# Autodesk Inventor assembly: servo grab
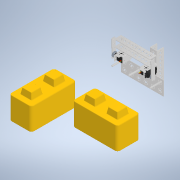
[picture p0: Inventor's stored thumbnail of the model, 180x180]
Saved by Autodesk Inventor 2020 (Build 240168000, 168)
## iProperties
Created: 2019-09-14
Part Number: servo grab
Document SubType Name: Assembly
Designer: tbloo
Author: tbloo
## Documents named in this file (9)
- D:\Documents\GitHub\AO_Robotics\CAD\Projects\Timothy Bloot\servo grab.iam
- D:\Documents\GitHub\AO_Robotics\CAD\Parts Kits\FTC Tetrix KOP Organized (7-24-19)\Stand-off posts\Tetrix_39103.ipt
- D:\Documents\GitHub\AO_Robotics\CAD\Parts Kits\FTC Tetrix KOP Organized (7-24-19)\Frame Hardware\Tetrix_39073.ipt
- D:\Documents\GitHub\AO_Robotics\CAD\Skystone Field\1x2 Block v2.ipt
- D:\Documents\GitHub\AO_Robotics\CAD\Parts Kits\FTC Tetrix KOP Organized (7-24-19)\Servo\Tetrix_39060.ipt
- D:\Documents\GitHub\AO_Robotics\CAD\Parts Kits\FTC Tetrix KOP Organized (7-24-19)\Servo\Tetrix_39197_Servo.ipt
- D:\Documents\GitHub\AO_Robotics\CAD\Parts Kits\FTC Tetrix KOP Organized (7-24-19)\Frame Hardware\Tetrix_39067.ipt
- D:\Documents\GitHub\AO_Robotics\CAD\Projects\Timothy Bloot\Tetrix_3907-5.ipt
- D:\Documents\GitHub\AO_Robotics\CAD\Parts Kits\FTC Tetrix KOP Organized (7-24-19)\Servo\Tetrix_39197_Metal_Horn.ipt
## Components (16 placed, 8 different names)
1. Tetrix_39103:1 — Rigid:8
2. Tetrix_39103:2 — Rigid:2
3. Tetrix_39103:3 — Rigid:1
4. Tetrix_39073:1 — Rigid:1, Rigid:2, Rigid:8, Rigid:9
5. 1x2 Block v2:1
6. Tetrix_39060:1 — Rigid:7, Rigid:17
7. Tetrix_39197_Servo:1 — Rigid:7, Rotational:1
8. 1x2 Block v2:2
9. Tetrix_39067:2 — Rigid:9, Rigid:19
10. Tetrix_39060:2 — Rigid:11, Rigid:16
11. Tetrix_39197_Servo:2 — Rigid:11, Rotational:2
12. Tetrix_39197_Metal_Horn:1 — Rotational:1, Rigid:14
13. Tetrix_39197_Metal_Horn:2 — Rotational:2, Rigid:15
14. Tetrix_3907-5:1 — Rigid:14, Cylindrical:1
15. Tetrix_3907-5:2 — Rigid:15, Cylindrical:1
16. Tetrix_39067:3 — Rigid:16, Rigid:17, Rigid:19
## Relationships (14: WeldJoint 11, RevoluteJoint 2, CylindricalJoint 1)
- Rigid:1 [WeldJoint]: Tetrix_39103:3 ↔ Tetrix_39073:1
- Rigid:2 [WeldJoint]: Tetrix_39103:2 ↔ Tetrix_39073:1
- Rigid:7 [WeldJoint]: Tetrix_39060:1 ↔ Tetrix_39197_Servo:1
- Rigid:8 [WeldJoint]: Tetrix_39103:1 ↔ Tetrix_39073:1
- Rigid:9 [WeldJoint]: Tetrix_39073:1 ↔ Tetrix_39067:2
- Rigid:11 [WeldJoint]: Tetrix_39060:2 ↔ Tetrix_39197_Servo:2
- Rotational:1 [RevoluteJoint]: Tetrix_39197_Servo:1 ↔ Tetrix_39197_Metal_Horn:1
- Rotational:2 [RevoluteJoint]: Tetrix_39197_Servo:2 ↔ Tetrix_39197_Metal_Horn:2
- Rigid:14 [WeldJoint]: Tetrix_39197_Metal_Horn:1 ↔ Tetrix_3907-5:1
- Rigid:15 [WeldJoint]: Tetrix_39197_Metal_Horn:2 ↔ Tetrix_3907-5:2
- Cylindrical:1: Tetrix_3907-5:1 ↔ Tetrix_3907-5:2
- Rigid:16 [WeldJoint]: Tetrix_39060:2 ↔ Tetrix_39067:3
- Rigid:17 [WeldJoint]: Tetrix_39060:1 ↔ Tetrix_39067:3
- Rigid:19 [WeldJoint]: Tetrix_39067:2 ↔ Tetrix_39067:3
